# Autodesk Inventor assembly: mount_04
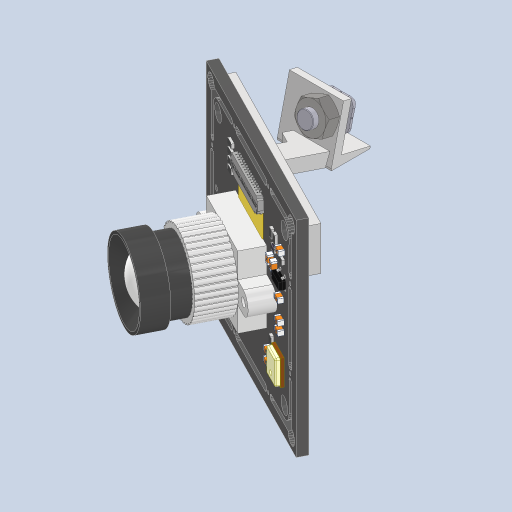
[picture p0: Inventor's stored thumbnail of the model, 512x512]
Saved by Autodesk Inventor 2024.4 (Build 284460000, 460)
## iProperties
Created: 2026-04-06
Part Number: mount_04
Document SubType Name: Assembly
Designer: tooles01
Author: tooles01
## Documents named in this file (5)
- C:\Users\tooles01\NYU Langone Health Dropbox\Shannon Toole\Shannon_Dropbox\Mar lab\RFID\CAD\Camera_mount_angled\mount_04.iam
- C:\Users\tooles01\NYU Langone Health Dropbox\Shannon Toole\Shannon_Dropbox\Mar lab\Inventor_Lib\Arducam OV9281.iam
- C:\Users\tooles01\NYU Langone Health Dropbox\Shannon Toole\Shannon_Dropbox\Mar lab\Inventor_Lib\100359 M3 BO SQUARE 6.ipt
- C:\Users\tooles01\Documents\Inventor\Content Center Files\R2024\en-US\AS 1112 (2)\AS 1112 - M3  Type 5.ipt
- C:\Users\tooles01\NYU Langone Health Dropbox\Shannon Toole\Shannon_Dropbox\Mar lab\RFID\CAD\Camera_mount_angled\angle_04.ipt
## Components (4 placed, 4 different names)
1. Arducam OV9281:1 [sub-assembly] — cam screw:1, cam screw:2
2. angle_04:1 — cam screw:1, cam screw:2, screw to angle piece:1, screw to angle piece:2, nut flush to angle piece
3. 100359 M3 BO SQUARE 6:1 — screw to angle piece:1, nut to screw:1, screw to angle piece:2
4. AS 1112 (2) - Metric M3  Type 5:1 — nut flush to angle piece, nut to screw:1
## Relationships (6: Mate 4, Insert 2)
- cam screw:1 [Insert]: Arducam OV9281:1 ↔ angle_04:1
- cam screw:2 [Insert]: Arducam OV9281:1 ↔ angle_04:1
- screw to angle piece:1 [Mate]: angle_04:1 ↔ 100359 M3 BO SQUARE 6:1
- screw to angle piece:2 [Mate] (-1 mm): angle_04:1 ↔ 100359 M3 BO SQUARE 6:1
- nut flush to angle piece [Mate]: angle_04:1 ↔ AS 1112 (2) - Metric M3  Type 5:1
- nut to screw:1 [Mate]: 100359 M3 BO SQUARE 6:1 ↔ AS 1112 (2) - Metric M3  Type 5:1
